# Autodesk Inventor assembly: BrueckenGR_LVE2560E
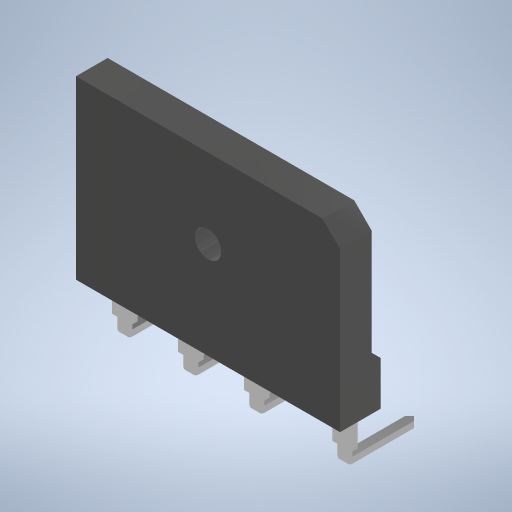
[picture p0: Inventor's stored thumbnail of the model, 512x512]
Saved by Autodesk Inventor 2023.1 (Build 271208000, 208)
## iProperties
Created: 2023-11-19
Part Number: BrueckenGR_LVE2560E
Document SubType Name: Assembly
Designer: JansenL
Author: JansenL
## Documents named in this file (3)
- C:\Users\JansenL\Documents\FHM\Semester_1\ProjektMech\CAD-files\BrueckenGR_LVE2560E.iam
- C:\Users\JansenL\Documents\FHM\Semester_1\ProjektMech\CAD-files\BrueckenGR_LVE2560E.ipt
- C:\Users\JansenL\Documents\FHM\Semester_1\ProjektMech\CAD-files\BrueckenGR_LVE2560E_Feet.ipt
## Components (5 placed, 2 different names)
1. BrueckenGR_LVE2560E:1 — Mate:1, Flush:5, Mate:6, Flush:9, Mate:7, Flush:10, Mate:10
2. BrueckenGR_LVE2560E_Feet:1 — Mate:1, Flush:5, Flush:10, Flush:11, Flush:12, Flush:13, Flush:18
3. BrueckenGR_LVE2560E_Feet:2 — Flush:11, Flush:14, Flush:15, Flush:16, Flush:18, Mate:10
4. BrueckenGR_LVE2560E_Feet:3 — Flush:12, Flush:14, Flush:16, Flush:17
5. BrueckenGR_LVE2560E_Feet:4 — Flush:13, Flush:15, Flush:17
## Relationships (15: Flush 11, Mate 4)
- Mate:1: BrueckenGR_LVE2560E:1 ↔ BrueckenGR_LVE2560E_Feet:1
- Flush:5 (-2.5 mm): BrueckenGR_LVE2560E:1 ↔ BrueckenGR_LVE2560E_Feet:1
- Mate:6: BrueckenGR_LVE2560E:1
- Flush:9: BrueckenGR_LVE2560E:1
- Mate:7: BrueckenGR_LVE2560E:1
- Flush:10 (2.7 mm): BrueckenGR_LVE2560E:1 ↔ BrueckenGR_LVE2560E_Feet:1
- Flush:11: BrueckenGR_LVE2560E_Feet:1 ↔ BrueckenGR_LVE2560E_Feet:2
- Flush:12: BrueckenGR_LVE2560E_Feet:1 ↔ BrueckenGR_LVE2560E_Feet:3
- Flush:13: BrueckenGR_LVE2560E_Feet:1 ↔ BrueckenGR_LVE2560E_Feet:4
- Flush:14: BrueckenGR_LVE2560E_Feet:2 ↔ BrueckenGR_LVE2560E_Feet:3
- Flush:15: BrueckenGR_LVE2560E_Feet:2 ↔ BrueckenGR_LVE2560E_Feet:4
- Flush:16 (-7.5 mm): BrueckenGR_LVE2560E_Feet:2 ↔ BrueckenGR_LVE2560E_Feet:3
- Flush:17 (-7.5 mm): BrueckenGR_LVE2560E_Feet:3 ↔ BrueckenGR_LVE2560E_Feet:4
- Flush:18 (-10 mm): BrueckenGR_LVE2560E_Feet:1 ↔ BrueckenGR_LVE2560E_Feet:2
- Mate:10: BrueckenGR_LVE2560E:1 ↔ BrueckenGR_LVE2560E_Feet:2
